# Autodesk Inventor assembly: CL7-100
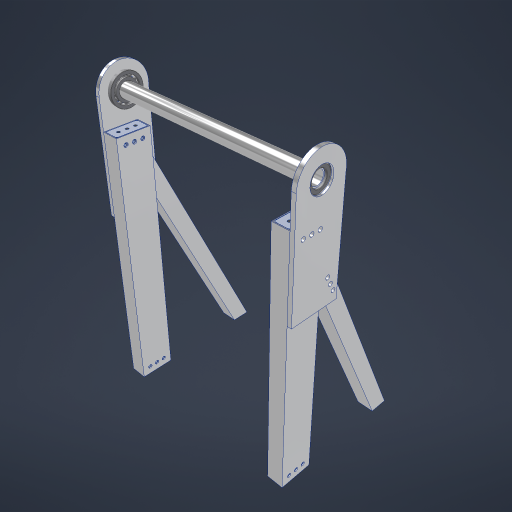
[picture p0: Inventor's stored thumbnail of the model, 512x512]
Saved by Autodesk Inventor 2023.4 (Build 274418000, 418)
## iProperties
Created: 2025-03-17
Part Number: CL7-100
Document SubType Name: Assembly
Designer: dlangdon
Author: dlangdon
## Documents named in this file (7)
- C:\Users\brand\OneDrive\Documents\GitHub\robotics 23\2025-ReefScape---CAD\Climber\CL7\CL7-100.iam
- C:\Users\brand\OneDrive\Documents\GitHub\robotics 23\2025-ReefScape---CAD\Climber\CL7\CL7-001.ipt
- C:\Users\brand\OneDrive\Documents\GitHub\robotics 23\2025-ReefScape---CAD\Climber\CL7\CL-002.ipt
- C:\Users\brand\OneDrive\Documents\GitHub\robotics 23\2025-ReefScape---CAD\Climber\CL7\CL7-003.ipt
- C:\Users\brand\OneDrive\Documents\GitHub\robotics 23\2025-ReefScape---CAD\COMMON PARTS\BEARINGS\0_875_ID_1_875OD_0_375_Thick60355K508_Ball Bearing.ipt
- C:\Users\brand\OneDrive\Documents\GitHub\robotics 23\2025-ReefScape---CAD\Elevator\EL2\EL2-005.ipt
- C:\Users\brand\OneDrive\Documents\GitHub\robotics 23\2025-ReefScape---CAD\Climber\CL7\CL7-007.ipt
## Components (13 placed, 6 different names)
1. CL7-001:1 — Flush:1, Flush:2, Mate:1, Mate:2, Flush:3, Flush:4, Insert:3, Insert:4, Insert:7, Insert:8, Insert:11, Insert:12
2. CL7-001:2 — Flush:1, Flush:2, Mate:1, Mate:3, Flush:5, Flush:6, Insert:1, Insert:2, Insert:5, Insert:6, Insert:9, Insert:10
3. CL-002:1 — Mate:2, Flush:3, Flush:4
4. CL-002:2 — Mate:3, Flush:5, Flush:6
5. CL7-003:1 — Mate:4, Mate:5
6. 0_875_ID_1_875OD_0_375_Thick60355K508_Ball Bearing:1 — Mate:4, Symmetry:1, Insert:13
7. 0_875_ID_1_875OD_0_375_Thick60355K508_Ball Bearing:2 — Mate:5, Symmetry:1, Insert:14
8. EL2-005:1 — Insert:1, Insert:2
9. EL2-005:2 — Insert:3, Insert:4
10. EL2-005:3 — Insert:5, Insert:6
11. EL2-005:4 — Insert:7, Insert:8
12. CL7-007:1 — Insert:11, Insert:12, Insert:13
13. CL7-007:2 — Insert:9, Insert:10, Insert:14
## Relationships (26: Insert 14, Flush 6, Mate 5, Symmetry 1)
- Flush:1: CL7-001:1 ↔ CL7-001:2
- Flush:2: CL7-001:1 ↔ CL7-001:2
- Mate:1 (254 mm): CL7-001:1 ↔ CL7-001:2
- Mate:2: CL7-001:1 ↔ CL-002:1
- Flush:3: CL7-001:1 ↔ CL-002:1
- Flush:4: CL7-001:1 ↔ CL-002:1
- Mate:3: CL7-001:2 ↔ CL-002:2
- Flush:5: CL7-001:2 ↔ CL-002:2
- Flush:6: CL7-001:2 ↔ CL-002:2
- Mate:4: CL7-003:1 ↔ 0_875_ID_1_875OD_0_375_Thick60355K508_Ball Bearing:1
- Mate:5: CL7-003:1 ↔ 0_875_ID_1_875OD_0_375_Thick60355K508_Ball Bearing:2
- Symmetry:1: 0_875_ID_1_875OD_0_375_Thick60355K508_Ball Bearing:1 ↔ 0_875_ID_1_875OD_0_375_Thick60355K508_Ball Bearing:2
- Insert:1: CL7-001:2 ↔ EL2-005:1
- Insert:2: CL7-001:2 ↔ EL2-005:1
- Insert:3: CL7-001:1 ↔ EL2-005:2
- Insert:4: CL7-001:1 ↔ EL2-005:2
- Insert:5: CL7-001:2 ↔ EL2-005:3
- Insert:6: CL7-001:2 ↔ EL2-005:3
- Insert:7: CL7-001:1 ↔ EL2-005:4
- Insert:8: CL7-001:1 ↔ EL2-005:4
- Insert:9: CL7-001:2 ↔ CL7-007:2
- Insert:10: CL7-001:2 ↔ CL7-007:2
- Insert:11: CL7-001:1 ↔ CL7-007:1
- Insert:12: CL7-001:1 ↔ CL7-007:1
- Insert:13: 0_875_ID_1_875OD_0_375_Thick60355K508_Ball Bearing:1 ↔ CL7-007:1
- Insert:14: 0_875_ID_1_875OD_0_375_Thick60355K508_Ball Bearing:2 ↔ CL7-007:2
